# Autodesk Inventor assembly: Robot A
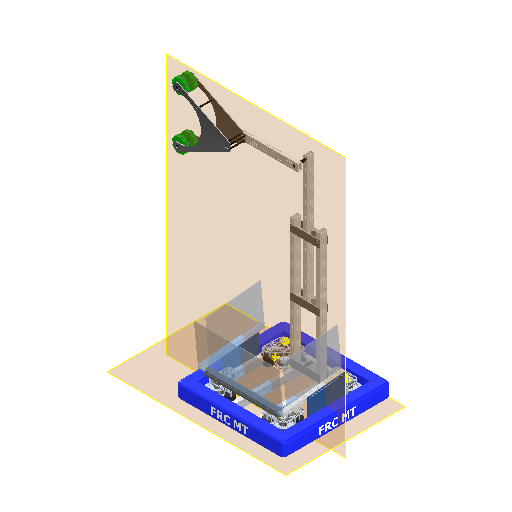
[picture p0: Inventor's stored thumbnail of the model, 512x512]
Saved by Autodesk Inventor 2025.3 (Build 293356000, 356)
## iProperties
Created: 2026-05-20
Part Number: Robot A
Document SubType Name: Assembly
Designer: djair.oliveira
Author: djair.oliveira
## Documents named in this file (6)
- C:\Users\djair.oliveira\Documents\GitHub\MT_2026\CAD\Model A\Robot A.iam
- C:\Users\djair.oliveira\Documents\GitHub\MT_2026\CAD\Model A\Chassi\Chassi.iam
- C:\Users\djair.oliveira\Documents\GitHub\MT_2026\CAD\Model A\Intake\Intake.iam
- C:\Users\djair.oliveira\Documents\GitHub\MT_2026\CAD\Model A\Bumper.ipt
- C:\Users\djair.oliveira\Documents\GitHub\MT_2026\CAD\Model A\Elevador\Elevador.iam
- C:\Users\djair.oliveira\Documents\GitHub\MT_2026\CAD\Model A\Hand\Hand.iam
## Components (5 placed, 5 different names)
1. Chassi:1 [sub-assembly] — Alinhado:1, Alinhado:2, Alinhado:3, Coincidente:1, Coincidente:2, Coincidente:3, Coincidente:5, Coincidente:6, Alinhado:4, Alinhado:5
2. Intake:1 [sub-assembly] — Coincidente:1, Coincidente:2, Coincidente:3, Coincidente:4
3. Bumper:1 — Coincidente:4, Coincidente:5
4. Elevador:1 [sub-assembly] — Coincidente:6, Alinhado:4, Alinhado:5, Coincidente:7, Alinhado:6
5. Hand:1 [sub-assembly] — Coincidente:7, Alinhado:6
## Relationships (13: Mate 7, Flush 6)
- Alinhado:1 [Flush]: Chassi:1
- Alinhado:2 [Flush]: Chassi:1
- Alinhado:3 [Flush]: Chassi:1
- Coincidente:1 [Mate]: Chassi:1 ↔ Intake:1
- Coincidente:2 [Mate]: Chassi:1 ↔ Intake:1
- Coincidente:3 [Mate]: Chassi:1 ↔ Intake:1
- Coincidente:4 [Mate] (1 mm): Intake:1 ↔ Bumper:1
- Coincidente:5 [Mate] (5 mm): Chassi:1 ↔ Bumper:1
- Coincidente:6 [Mate]: Chassi:1 ↔ Elevador:1
- Alinhado:4 [Flush]: Chassi:1 ↔ Elevador:1
- Alinhado:5 [Flush] (-88.9 mm): Chassi:1 ↔ Elevador:1
- Coincidente:7 [Mate]: Elevador:1 ↔ Hand:1
- Alinhado:6 [Flush]: Elevador:1 ↔ Hand:1
